# Autodesk Inventor assembly: МПСТ Редуктор
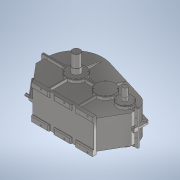
[picture p0: Inventor's stored thumbnail of the model, 180x180]
Saved by Autodesk Inventor 2022.1 (Build 261234020, 234B)
## iProperties
Created: 2021-09-16
Part Number: МПСТ Редуктор
Document SubType Name: Assembly
Designer: Алексанян Г.
Author: Алексанян Г.
## Documents named in this file (24)
- C:\Users\Гарник\Desktop\учёба\5 семак\Детмаш\Reductor\МПСТ Редуктор.iam
- C:\Users\Гарник\Desktop\учёба\5 семак\Детмаш\Reductor\МПСТ Промежуточный Вал.iam
- C:\Users\Гарник\Desktop\учёба\5 семак\Детмаш\Reductor\МПСТ Быстроходный Вал.iam
- C:\Users\Гарник\Desktop\учёба\5 семак\Детмаш\Reductor\МПСТ Редуктор\Мастер проектирования\Цилиндрическое зубчатое зацепление11.ipt
- C:\Users\Гарник\Desktop\учёба\5 семак\Детмаш\Reductor\МПСТ Шпонка переходного вала.ipt
- C:\Users\Гарник\Desktop\учёба\5 семак\Детмаш\Reductor\МПСТ Редуктор\Мастер проектирования\Цилиндрическое зубчатое зацепление12.ipt
- C:\Users\Гарник\Desktop\учёба\5 семак\Детмаш\Reductor\МПСТ Редуктор\Мастер проектирования\Подшипник1.iam
- C:\Users\Гарник\Desktop\учёба\5 семак\Детмаш\Reductor\МПСТ Редуктор\Мастер проектирования\Подшипник2.iam
- C:\Users\Гарник\Desktop\учёба\5 семак\Детмаш\Reductor\МПСТ Редуктор\Мастер проектирования\Подшипник5.iam
- C:\Users\Гарник\Desktop\учёба\5 семак\Детмаш\Reductor\МПСТ Редуктор\Мастер проектирования\Подшипник6.iam
- C:\Users\Гарник\Desktop\учёба\5 семак\Детмаш\Reductor\МПСТ Корпус.ipt
- C:\Users\Гарник\Desktop\учёба\5 семак\Детмаш\Reductor\МПСТ Крышка подшипника глухая 110.ipt
- C:\Users\Гарник\Desktop\учёба\5 семак\Детмаш\Reductor\МПСТ Крышка подшипника с отверстием 110.ipt
- C:\Users\Гарник\Desktop\учёба\5 семак\Детмаш\Reductor\МПСТ Крышка подшипника глухая 150.ipt
- C:\Users\Гарник\Desktop\учёба\5 семак\Детмаш\Reductor\МПСТ Редуктор\Мастер проектирования\Цилиндрическое зубчатое зацепление22.ipt
- C:\Users\Гарник\Desktop\учёба\5 семак\Детмаш\Reductor\МПСТ Мазеудерживающее кольцо быстроходного вала.ipt
- C:\Users\Гарник\Desktop\учёба\5 семак\Детмаш\Reductor\МПСТ Тихоходный Вал.iam
- C:\Users\Гарник\Desktop\учёба\5 семак\Детмаш\Reductor\МПСТ Шпонка тихоходного вала.ipt
- C:\Users\Гарник\Desktop\учёба\5 семак\Детмаш\Reductor\МПСТ Редуктор\Мастер проектирования\Цилиндрическое зубчатое зацепление21.ipt
- C:\Users\Гарник\Desktop\учёба\5 семак\Детмаш\Reductor\МПСТ Крышка подшипника с отверстием 150.ipt
- C:\Users\Гарник\Desktop\учёба\5 семак\Детмаш\Reductor\МПСТ Редуктор\Мастер проектирования\Подшипник3.iam
- C:\Users\Гарник\Desktop\учёба\5 семак\Детмаш\Reductor\МПСТ Редуктор\Мастер проектирования\Подшипник4.iam
- C:\Users\Гарник\Desktop\учёба\5 семак\Детмаш\Reductor\МПСТ Крышка корпуса.ipt
- C:\Users\Гарник\Desktop\учёба\5 семак\Детмаш\Reductor\МПСТ Люк.ipt
## Components (26 placed, 16 different names)
1. МПСТ Корпус:1 — Совмещение:1, Вставка:2, Совмещение:2, Совмещение:3, Совмещение:8, Совмещение:9, Вставка:3, Вставка:4, Вставка:5, Вставка:6, Совмещение:11, Совмещение:12, Совмещение:13, Совмещение:14, Совмещение:15, Совмещение:16, Совмещение:17, Совмещение:28, Вставка:12, Совмещение:32, Совмещение:33, Совмещение:38, Совмещение:39, Совмещение:40
2. МПСТ Быстроходный Вал:1 [sub-assembly] — Совмещение:1, Вставка:1, Совмещение:4, Совмещение:5, Совмещение:7, Касательность:1, Совмещение:25, ЗубчПер:1
3. Цилиндрическое зубчатое зацепление1:1 — Вставка:1, ЗубчПер:1
4. МПСТ Крышка подшипника глухая 110:1 — Вставка:2, Совмещение:2, Совмещение:3, Совмещение:6
5. Подшипник:1 [sub-assembly] — Совмещение:4, Совмещение:5, Совмещение:6
6. Подшипник:2 [sub-assembly] — Совмещение:7, Совмещение:10
7. МПСТ Крышка подшипника с отверстием 110:1 — Совмещение:8, Совмещение:9, Вставка:3, Совмещение:10
8. МПСТ Крышка подшипника глухая 150:1 — Вставка:4, Совмещение:15, Совмещение:16, Совмещение:19
9. МПСТ Крышка подшипника глухая 150:2 — Вставка:5, Совмещение:13, Совмещение:14, Совмещение:36
10. МПСТ Крышка подшипника глухая 150:3 — Вставка:6, Совмещение:11, Совмещение:12, Совмещение:21
11. МПСТ Промежуточный Вал:1 [sub-assembly] — Совмещение:17, Совмещение:18, Совмещение:20, Вставка:7, Вставка:8, Вставка:9, Совмещение:22, Касательность:2, Совмещение:26, ЗубчПер:2
12. Подшипник:3 [sub-assembly] — Совмещение:20, Совмещение:21, Совмещение:27
13. Подшипник:4 [sub-assembly] — Совмещение:18, Совмещение:19
14. Цилиндрическое зубчатое зацепление1:2 — Вставка:9, Совмещение:24, Совмещение:27, ЗубчПер:2
15. МПСТ Шпонка переходного вала:1 — Вставка:7, Вставка:8, Совмещение:23
16. Цилиндрическое зубчатое зацепление2:1 — Совмещение:22, Совмещение:23, Совмещение:24
17. МПСТ Мазеудерживающее кольцо быстроходного вала:1 — Касательность:1, Совмещение:25
18. МПСТ Мазеудерживающее кольцо быстроходного вала:2 — Касательность:2, Совмещение:26
19. МПСТ Тихоходный Вал:1 [sub-assembly] — Совмещение:28, Вставка:10, Вставка:11, Совмещение:29, Совмещение:31, Совмещение:34, Совмещение:35
20. МПСТ Шпонка тихоходного вала:1 — Вставка:10, Вставка:11, Совмещение:30
21. Цилиндрическое зубчатое зацепление2:2 — Совмещение:29, Совмещение:30, Совмещение:31
22. МПСТ Крышка подшипника с отверстием 150:1 — Вставка:12, Совмещение:32, Совмещение:33, Совмещение:37
23. Подшипник:5 [sub-assembly] — Совмещение:35, Совмещение:36
24. Подшипник:6 [sub-assembly] — Совмещение:34, Совмещение:37
25. МПСТ Крышка корпуса:1 — Совмещение:38, Совмещение:39, Совмещение:40, Совмещение:41, Совмещение:42, Совмещение:43
26. МПСТ Люк:1 — Совмещение:41, Совмещение:42, Совмещение:43
## Relationships (59: Mate 43, Insert 12, Tangent 2, RelateRotation 2)
- Совмещение:1 [Mate]: МПСТ Корпус:1 ↔ МПСТ Быстроходный Вал:1
- Вставка:1 [Insert]: МПСТ Быстроходный Вал:1 ↔ Цилиндрическое зубчатое зацепление1:1
- Вставка:2 [Insert]: МПСТ Корпус:1 ↔ МПСТ Крышка подшипника глухая 110:1
- Совмещение:2 [Mate]: МПСТ Корпус:1 ↔ МПСТ Крышка подшипника глухая 110:1
- Совмещение:3 [Mate]: МПСТ Корпус:1 ↔ МПСТ Крышка подшипника глухая 110:1
- Совмещение:4 [Mate]: МПСТ Быстроходный Вал:1 ↔ Подшипник:1
- Совмещение:5 [Mate]: МПСТ Быстроходный Вал:1 ↔ Подшипник:1
- Совмещение:6 [Mate]: МПСТ Крышка подшипника глухая 110:1 ↔ Подшипник:1
- Совмещение:7 [Mate]: МПСТ Быстроходный Вал:1 ↔ Подшипник:2
- Совмещение:8 [Mate]: МПСТ Корпус:1 ↔ МПСТ Крышка подшипника с отверстием 110:1
- Совмещение:9 [Mate]: МПСТ Корпус:1 ↔ МПСТ Крышка подшипника с отверстием 110:1
- Вставка:3 [Insert]: МПСТ Корпус:1 ↔ МПСТ Крышка подшипника с отверстием 110:1
- Совмещение:10 [Mate]: Подшипник:2 ↔ МПСТ Крышка подшипника с отверстием 110:1
- Вставка:4 [Insert]: МПСТ Корпус:1 ↔ МПСТ Крышка подшипника глухая 150:1
- Вставка:5 [Insert]: МПСТ Корпус:1 ↔ МПСТ Крышка подшипника глухая 150:2
- Вставка:6 [Insert]: МПСТ Корпус:1 ↔ МПСТ Крышка подшипника глухая 150:3
- Совмещение:11 [Mate]: МПСТ Корпус:1 ↔ МПСТ Крышка подшипника глухая 150:3
- Совмещение:12 [Mate]: МПСТ Корпус:1 ↔ МПСТ Крышка подшипника глухая 150:3
- Совмещение:13 [Mate]: МПСТ Корпус:1 ↔ МПСТ Крышка подшипника глухая 150:2
- Совмещение:14 [Mate]: МПСТ Корпус:1 ↔ МПСТ Крышка подшипника глухая 150:2
- Совмещение:15 [Mate]: МПСТ Корпус:1 ↔ МПСТ Крышка подшипника глухая 150:1
- Совмещение:16 [Mate]: МПСТ Корпус:1 ↔ МПСТ Крышка подшипника глухая 150:1
- Совмещение:17 [Mate]: МПСТ Корпус:1 ↔ МПСТ Промежуточный Вал:1
- Совмещение:18 [Mate]: МПСТ Промежуточный Вал:1 ↔ Подшипник:4
- Совмещение:19 [Mate]: МПСТ Крышка подшипника глухая 150:1 ↔ Подшипник:4
- Совмещение:20 [Mate]: МПСТ Промежуточный Вал:1 ↔ Подшипник:3
- Совмещение:21 [Mate]: МПСТ Крышка подшипника глухая 150:3 ↔ Подшипник:3
- Вставка:7 [Insert]: МПСТ Промежуточный Вал:1 ↔ МПСТ Шпонка переходного вала:1
- Вставка:8 [Insert]: МПСТ Промежуточный Вал:1 ↔ МПСТ Шпонка переходного вала:1
- Вставка:9 [Insert]: МПСТ Промежуточный Вал:1 ↔ Цилиндрическое зубчатое зацепление1:2
- Совмещение:22 [Mate]: МПСТ Промежуточный Вал:1 ↔ Цилиндрическое зубчатое зацепление2:1
- Совмещение:23 [Mate]: МПСТ Шпонка переходного вала:1 ↔ Цилиндрическое зубчатое зацепление2:1
- Совмещение:24 [Mate]: Цилиндрическое зубчатое зацепление1:2 ↔ Цилиндрическое зубчатое зацепление2:1
- Касательность:1 [Tangent]: МПСТ Быстроходный Вал:1 ↔ МПСТ Мазеудерживающее кольцо быстроходного вала:1
- Совмещение:25 [Mate]: МПСТ Быстроходный Вал:1 ↔ МПСТ Мазеудерживающее кольцо быстроходного вала:1
- Касательность:2 [Tangent]: МПСТ Промежуточный Вал:1 ↔ МПСТ Мазеудерживающее кольцо быстроходного вала:2
- Совмещение:26 [Mate]: МПСТ Промежуточный Вал:1 ↔ МПСТ Мазеудерживающее кольцо быстроходного вала:2
- Совмещение:27 [Mate]: Подшипник:3 ↔ Цилиндрическое зубчатое зацепление1:2
- Совмещение:28 [Mate]: МПСТ Корпус:1 ↔ МПСТ Тихоходный Вал:1
- Вставка:10 [Insert]: МПСТ Тихоходный Вал:1 ↔ МПСТ Шпонка тихоходного вала:1
- Вставка:11 [Insert]: МПСТ Тихоходный Вал:1 ↔ МПСТ Шпонка тихоходного вала:1
- Совмещение:29 [Mate]: МПСТ Тихоходный Вал:1 ↔ Цилиндрическое зубчатое зацепление2:2
- Совмещение:30 [Mate]: МПСТ Шпонка тихоходного вала:1 ↔ Цилиндрическое зубчатое зацепление2:2
- Совмещение:31 [Mate]: МПСТ Тихоходный Вал:1 ↔ Цилиндрическое зубчатое зацепление2:2
- Вставка:12 [Insert]: МПСТ Корпус:1 ↔ МПСТ Крышка подшипника с отверстием 150:1
- Совмещение:32 [Mate]: МПСТ Корпус:1 ↔ МПСТ Крышка подшипника с отверстием 150:1
- Совмещение:33 [Mate]: МПСТ Корпус:1 ↔ МПСТ Крышка подшипника с отверстием 150:1
- Совмещение:34 [Mate]: МПСТ Тихоходный Вал:1 ↔ Подшипник:6
- Совмещение:35 [Mate]: МПСТ Тихоходный Вал:1 ↔ Подшипник:5
- Совмещение:36 [Mate]: МПСТ Крышка подшипника глухая 150:2 ↔ Подшипник:5
- Совмещение:37 [Mate]: МПСТ Крышка подшипника с отверстием 150:1 ↔ Подшипник:6
- ЗубчПер:1 [RelateRotation] (1 ul): МПСТ Быстроходный Вал:1 ↔ Цилиндрическое зубчатое зацепление1:1
- ЗубчПер:2 [RelateRotation] (1 ul): МПСТ Промежуточный Вал:1 ↔ Цилиндрическое зубчатое зацепление1:2
- Совмещение:38 [Mate]: МПСТ Корпус:1 ↔ МПСТ Крышка корпуса:1
- Совмещение:39 [Mate]: МПСТ Корпус:1 ↔ МПСТ Крышка корпуса:1
- Совмещение:40 [Mate]: МПСТ Корпус:1 ↔ МПСТ Крышка корпуса:1
- Совмещение:41 [Mate]: МПСТ Крышка корпуса:1 ↔ МПСТ Люк:1
- Совмещение:42 [Mate]: МПСТ Крышка корпуса:1 ↔ МПСТ Люк:1
- Совмещение:43 [Mate]: МПСТ Крышка корпуса:1 ↔ МПСТ Люк:1
